# Autodesk Inventor assembly: Tiger
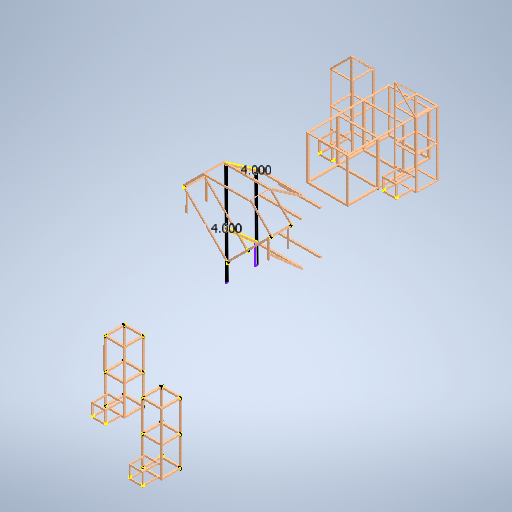
[picture p0: Inventor's stored thumbnail of the model, 512x512]
Saved by Autodesk Inventor 2025 (Build 290162000, 162)
## iProperties
Created: 2024-06-05
Part Number: Tiger
Document SubType Name: Assembly
Designer: Cupri
Mass: 180546 g
Surface Area: 136258 cm^2
Volume: 328266 cm^3
Density: 0.55 g/cm^3
Author: Cupri
## Documents named in this file (38)
- C:\Users\Win\Documents\GitHub\USCTigerBurn24\v2\Tiger.iam
- C:\Users\Win\Documents\GitHub\USCTigerBurn24\Standard Timber\4x4x72.ipt
- C:\Users\Win\Documents\GitHub\USCTigerBurn24\Standard Timber\4x4x40.ipt
- C:\Users\Win\Documents\GitHub\USCTigerBurn24\Standard Timber\2x4x36.ipt
- C:\Users\Win\Documents\GitHub\USCTigerBurn24\Standard Timber\2x4x40.ipt
- C:\Users\Win\Documents\GitHub\USCTigerBurn24\Standard Timber\2x4x24.ipt
- C:\Users\Win\Documents\GitHub\USCTigerBurn24\Standard Timber\2x4x28.ipt
- C:\Users\Win\Documents\GitHub\USCTigerBurn24\Standard Timber\2x4x72 (45 90).ipt
- C:\Users\Win\Documents\GitHub\USCTigerBurn24\Standard Timber\2x4x68 (45 90).ipt
- C:\Users\Win\Documents\GitHub\USCTigerBurn24\Standard Timber\2x4x42.343 (45 90).ipt
- C:\Users\Win\Documents\GitHub\USCTigerBurn24\Standard Timber\2x4x72 (30 90).ipt
- C:\Users\Win\Documents\GitHub\USCTigerBurn24\Standard Timber\2x4x44.ipt
- C:\Users\Win\Documents\GitHub\USCTigerBurn24\Standard Timber\4x4x104.303.ipt
- C:\Users\Win\Documents\GitHub\USCTigerBurn24\Standard Timber\4x4xigiveup.ipt
- C:\Users\Win\Documents\GitHub\USCTigerBurn24\Standard Timber\4x4x96.ipt
- C:\Users\Win\Documents\GitHub\USCTigerBurn24\Standard Timber\2x4x96.ipt
- C:\Users\Win\Documents\GitHub\USCTigerBurn24\Standard Timber\2x4xidk.ipt
- C:\Users\Win\Documents\GitHub\USCTigerBurn24\Standard Timber\2x4x120.ipt
- C:\Users\Win\Documents\GitHub\USCTigerBurn24\Standard Timber\2x4x72.ipt
- C:\Users\Win\Documents\GitHub\USCTigerBurn24\Standard Timber\2x4x88.ipt
- C:\Users\Win\Documents\GitHub\USCTigerBurn24\Standard Timber\4x4x55.ipt
- C:\Users\Win\Documents\GitHub\USCTigerBurn24\Standard Timber\4x4x66.ipt
- C:\Users\Win\Documents\GitHub\USCTigerBurn24\Standard Timber\2x4x48.ipt
- C:\Users\Win\Documents\GitHub\USCTigerBurn24\Standard Timber\leg slant.ipt
- C:\Users\Win\Documents\GitHub\USCTigerBurn24\Standard Timber\Leg slant.2.ipt
- C:\Users\Win\Documents\GitHub\USCTigerBurn24\Standard Timber\2x4x48_MIR.ipt
- C:\Users\Win\Documents\GitHub\USCTigerBurn24\Standard Timber\2x4x72_MIR.ipt
- C:\Users\Win\Documents\GitHub\USCTigerBurn24\Standard Timber\2x4x36_MIR.ipt
- C:\Users\Win\Documents\GitHub\USCTigerBurn24\Standard Timber\2x4x24_MIR.ipt
- C:\Users\Win\Documents\GitHub\USCTigerBurn24\Standard Timber\2x4x28_MIR.ipt
- C:\Users\Win\Documents\GitHub\USCTigerBurn24\Standard Timber\leg slant_MIR.ipt
- C:\Users\Win\Documents\GitHub\USCTigerBurn24\Standard Timber\Leg slant.2_MIR.ipt
- C:\Users\Win\Documents\GitHub\USCTigerBurn24\v2\Tiger\AIP\FEA\epzzwi8io.fins
- C:\Users\Win\Documents\GitHub\USCTigerBurn24\v2\Tiger\AIP\FEA\epzzwi8io.fsat
- C:\Users\Win\Documents\GitHub\USCTigerBurn24\v2\Tiger\AIP\FEA\epzzwi8io.ftes
- C:\Users\Win\Documents\GitHub\USCTigerBurn24\v2\Tiger\AIP\FEA\epzzwi8io.fwiz
- C:\Users\Win\Documents\GitHub\USCTigerBurn24\v2\Tiger\AIP\FEA\epzzwi8jk.fmsh
- C:\Users\Win\Documents\GitHub\USCTigerBurn24\v2\Tiger\AIP\FEA\epzzwi8jl.fres
## Components (186 placed, 31 different names)
1. 4x4x104.303:1 — Flush:221, Flush:222
2. 4x4x104.303:2 — Flush:221, Flush:222
3. 4x4xigiveup:1 — Mate:186
4. 4x4xigiveup:2 — Flush:237, Mate:187, Mate:188
5. 4x4x96:1 — Flush:232
6. 4x4x96:2 — Flush:232
7. 4x4x96:3 — Flush:230
8. 4x4x96:4 — Flush:230
9. 4x4x96:5
10. 2x4x96:1 — Mate:186, Flush:237, Mate:187, Mate:188, Mate:191
11. 2x4xidk:1 — Mate:189, Mate:190, Mate:191, Flush:241
12. 2x4xidk:2 — Mate:192, Flush:240, Flush:241
13. 2x4x72 (45 90):1 — Flush:88
14. 2x4x68 (45 90):1 — Flush:44, Flush:88
15. 2x4x72 (45 90):2 — Flush:48, Mate:48, Flush:51, Mate:49
16. 2x4x72 (45 90):3 — Flush:44, Mate:45, Mate:50, Flush:52, Mate:51
17. 2x4x42.343 (45 90):1 — Flush:48
18. 2x4x42.343 (45 90):2 — Mate:45
19. 2x4x72 (30 90):1 — Mate:48, Flush:51, Mate:49, Flush:70, Flush:238, Mate:192, Flush:240
20. 2x4x72 (30 90):2 — Mate:50, Flush:52, Mate:51, Flush:71, Flush:72
21. 2x4x72 (45 90):4 — Mate:61, Flush:61, Flush:62
22. 2x4x68 (45 90):2 — Mate:61, Flush:61, Flush:62
23. 2x4x72 (45 90):5 — Flush:59, Mate:59, Mate:65, Flush:67, Flush:68
24. 2x4x72 (45 90):6 — Flush:63, Flush:64, Mate:68, Flush:73
25. 2x4x42.343 (45 90):3 — Flush:59, Mate:59
26. 2x4x42.343 (45 90):4 — Flush:63
27. 2x4x72 (30 90):3 — Mate:66, Flush:69, Flush:204, Mate:189
28. 2x4x72 (30 90):4 — Flush:64, Mate:67, Mate:69, Flush:239
29. 2x4x44:1 — Mate:67, Flush:71, Flush:72, Flush:239, Mate:190
30. 2x4x44:2 — Mate:65, Flush:67, Flush:68
31. 2x4x44:3 — Mate:66, Flush:69, Flush:70, Flush:204, Flush:238
32. 2x4x44:4 — Mate:68, Flush:73, Mate:69
33. 4x4x72:65
34. 4x4x72:66
35. 4x4x40:117
36. 4x4x40:118
37. 4x4x40:119
38. 4x4x40:120
39. 4x4x40:121
40. 4x4x40:122
41. 4x4x40:123
42. 4x4x40:124
43. 4x4x72:67
44. 4x4x72:68
45. 4x4x40:125
46. 4x4x40:126
47. 4x4x40:127
48. 2x4x40:7
49. 2x4x36:25
50. 2x4x36:26
51. 2x4x36:27
52. 2x4x36:28
53. 2x4x24:13
54. 2x4x24:14
55. 2x4x28:13
56. 2x4x28:14
57. 4x4x72:69
58. 4x4x72:70
59. 4x4x40:128
60. 4x4x40:129
61. 4x4x40:130
62. 4x4x40:131
63. 4x4x72:71
64. 4x4x72:72
65. 4x4x72:73
66. 4x4x72:74
67. 4x4x40:132
68. 4x4x40:133
69. 4x4x40:134
70. 4x4x40:135
71. 4x4x40:136
72. 4x4x40:137
73. 4x4x40:138
74. 4x4x40:139
75. 4x4x72:75
76. 4x4x72:76
77. 4x4x40:140
78. 4x4x40:141
79. 4x4x40:142
80. 2x4x40:8
81. 2x4x36:29
82. 2x4x36:30
83. 2x4x36:31
84. 2x4x36:32
85. 2x4x24:15
86. 2x4x24:16
87. 2x4x28:15
88. 2x4x28:16
89. 4x4x72:77
90. 4x4x72:78
91. 4x4x40:143
92. 4x4x40:144
93. 4x4x40:145
94. 4x4x40:146
95. 4x4x72:79
96. 4x4x72:80
97. 4x4x96:6 — Mate:293, Flush:350, Flush:351, Mate:301, Flush:367, Flush:368, Flush:390, Flush:528
98. 4x4x96:7 — Mate:293, Flush:350, Flush:351, Mate:294, Flush:352, Flush:353, Flush:393, Mate:316, Flush:405, Mate:318
99. 4x4x96:8 — Mate:294, Flush:352, Flush:353, Flush:365, Flush:366, Mate:300, Flush:531
100. 4x4x96:9 — Flush:361, Flush:362, Mate:298, Flush:384
101. 4x4x96:10 — Flush:396, Mate:314, Flush:397, Flush:399
102. 4x4x96:11 — Flush:363, Mate:299, Flush:364, Flush:398
103. 2x4x120:4 — Flush:361, Flush:362, Mate:298, Mate:301, Flush:367, Flush:368, Mate:303, Flush:371, Flush:372, Flush:383, Mate:309, Flush:385, Mate:310, Flush:386, Flush:387, Mate:311, Flush:389, Mate:312
104. 2x4x120:5 — Flush:363, Mate:299, Flush:364, Flush:365, Flush:366, Mate:300, Mate:302, Flush:369, Flush:370
105. 2x4x72:1 — Mate:302, Flush:369, Flush:370
106. 2x4x72:2 — Mate:303, Flush:371, Flush:372, Mate:306, Flush:377, Flush:378, Flush:391, Mate:313
107. 4x4x96:12 — Mate:306, Flush:377, Flush:378, Flush:392
108. 4x4x96:13 — Flush:403, Flush:404, Flush:406, Mate:317
109. 4x4x96:14
110. 4x4x96:15 — Flush:383, Mate:309, Flush:384, Mate:383
111. 4x4x96:16 — Flush:394, Flush:395, Mate:315, Flush:400, Flush:401
112. 4x4x96:17 — Flush:388
113. 2x4x88:1 — Flush:385, Mate:310, Flush:386
114. 2x4x88:2 — Flush:387, Mate:311, Flush:388
115. 2x4x88:3 — Flush:389, Flush:390, Mate:312
116. 2x4x88:4 — Flush:391, Flush:392, Mate:313
117. 4x4x55:1 — Flush:393, Flush:394, Flush:395
118. 4x4x55:2 — Flush:396, Mate:314, Flush:397, Flush:527
119. 4x4x55:3 — Flush:398, Flush:399, Mate:315, Flush:530
120. 4x4x55:4 — Flush:400, Mate:316, Flush:401, Mate:389
121. 4x4x66:1 — Flush:403, Flush:404, Mate:318
122. 4x4x66:2 — Flush:405, Flush:406, Mate:317
123. 2x4x48:1 — Mate:319, Flush:407, Flush:408, Mate:322, Mate:330, Flush:422, Flush:423
124. 2x4x48:2 — Flush:409, Mate:320, Flush:410, Mate:321, Flush:411, Mate:328, Flush:419, Flush:461, Mate:347, Flush:527
125. 2x4x48:3 — Mate:319, Flush:407, Flush:408, Flush:409, Mate:320, Flush:410, Mate:327, Flush:417, Flush:418
126. 2x4x48:4 — Mate:321, Flush:411, Mate:322, Mate:329, Flush:420, Flush:421
127. 2x4x48:5 — Flush:452
128. 2x4x48:6 — Flush:426, Flush:427
129. 2x4x48:7 — Mate:331, Flush:424, Flush:425, Flush:430, Flush:431, Flush:453, Mate:339
130. 2x4x48:8 — Flush:428, Flush:429
131. 2x4x72:3 — Mate:327, Flush:417, Flush:418, Mate:331, Flush:424, Flush:425, Flush:430, Flush:431
132. 2x4x72:4 — Mate:328, Flush:419, Flush:426, Flush:427, Mate:346, Flush:462
133. 2x4x72:5 — Mate:329, Flush:420, Flush:421, Flush:428, Flush:429, Flush:464, Mate:383
134. 2x4x72:6 — Mate:330, Flush:422, Flush:423
135. 2x4x48:9 — Flush:445, Flush:446
136. 2x4x48:10 — Mate:337, Flush:449, Flush:450
137. 2x4x48:11
138. 2x4x48:12 — Flush:447, Flush:448, Mate:338, Mate:349, Flush:465, Flush:466
139. 2x4x72:7 — Flush:452, Flush:453, Mate:339
140. 2x4x72:8 — Mate:337, Flush:449, Flush:450
141. 2x4x72:9 — Flush:447, Flush:448, Flush:451, Mate:338
142. 2x4x72:10 — Flush:445, Flush:446, Flush:451
143. 2x4x36:33
144. 2x4x36:34 — Flush:463, Flush:464
145. 2x4x36:35 — Mate:348, Mate:390
146. 2x4x36:36 — Flush:461, Mate:347
147. 2x4x24:17 — Flush:528
148. 2x4x24:18 — Mate:390
149. 2x4x28:17
150. 2x4x28:18
151. 2x4x48:13 — Mate:346, Flush:462, Mate:348, Flush:463
152. 2x4x48:14 — Mate:349, Flush:465, Flush:466, Flush:467, Flush:468, Flush:469, Flush:470
153. leg slant:1 — Flush:467, Flush:468
154. Leg slant.2:1 — Flush:469, Flush:470
155. 2x4x48_MIR:1 — Flush:473, Flush:474, Mate:351, Mate:352, Flush:494, Flush:495, Mate:362
156. 2x4x48_MIR:2 — Flush:471, Mate:350, Flush:472, Flush:475, Mate:353, Flush:489, Mate:360, Mate:371, Flush:519
157. 2x4x48_MIR:3 — Flush:471, Mate:350, Flush:472, Flush:473, Flush:474, Mate:351, Flush:485, Flush:486, Mate:359
158. 2x4x48_MIR:4 — Mate:352, Flush:475, Mate:353, Flush:492, Flush:493, Mate:361, Flush:530
159. 2x4x48_MIR:5 — Flush:477, Flush:479, Mate:355, Mate:356, Flush:502
160. 2x4x48_MIR:6 — Mate:354, Flush:476, Flush:478, Flush:480, Mate:357, Flush:487, Flush:488
161. 2x4x48_MIR:7 — Mate:354, Flush:476, Flush:477, Flush:478, Flush:479, Mate:355, Flush:481, Flush:482, Flush:483, Flush:484, Mate:358, Mate:367, Flush:501
162. 2x4x48_MIR:8 — Mate:356, Flush:480, Mate:357, Flush:490, Flush:491
163. 2x4x72_MIR:1 — Flush:481, Flush:482, Flush:483, Flush:484, Mate:358, Flush:485, Flush:486, Mate:359
164. 2x4x72_MIR:2 — Flush:487, Flush:488, Flush:489, Mate:360, Flush:524, Mate:377
165. 2x4x72_MIR:3 — Flush:490, Flush:491, Flush:492, Flush:493, Mate:361, Flush:518, Mate:389
166. 2x4x72_MIR:4 — Flush:494, Flush:495, Mate:362
167. 2x4x48_MIR:9 — Flush:497, Flush:499, Mate:364, Mate:365, Flush:516, Flush:517, Mate:391
168. 2x4x48_MIR:10 — Mate:363, Flush:496, Flush:498, Flush:500, Mate:366, Flush:507, Flush:508, Mate:369, Flush:509, Flush:510, Flush:529, Mate:387
169. 2x4x48_MIR:11 — Mate:363, Flush:496, Flush:497, Flush:498, Flush:499, Mate:364, Flush:503, Flush:504, Flush:505, Mate:368, Flush:506
170. 2x4x48_MIR:12 — Mate:365, Flush:500, Mate:366, Mate:370, Flush:511, Flush:512, Flush:513, Flush:514, Flush:525, Flush:526, Mate:378
171. 2x4x72_MIR:5 — Mate:367, Flush:501, Flush:502, Flush:503, Flush:504, Flush:505, Mate:368, Flush:506
172. 2x4x72_MIR:6 — Flush:507, Flush:508, Mate:369, Flush:509, Flush:510
173. 2x4x72_MIR:7 — Mate:370, Flush:511, Flush:512, Flush:513, Flush:514, Flush:515
174. 2x4x72_MIR:8 — Flush:515, Flush:516, Flush:517
175. 2x4x36_MIR:1 — Flush:522, Mate:375, Rigid:233
176. 2x4x36_MIR:2 — Flush:518, Mate:373, Flush:520, Mate:374, Flush:521, Flush:523
177. 2x4x36_MIR:3 — Mate:372, Mate:376, Rigid:235, Mate:388
178. 2x4x36_MIR:4 — Mate:371, Flush:519, Mate:372, Rigid:234, Rigid:236
179. 2x4x24_MIR:1 — Mate:373, Flush:520, Rigid:233, Flush:531
180. 2x4x24_MIR:2 — Rigid:234, Mate:388
181. 2x4x28_MIR:1 — Mate:374, Flush:521, Rigid:235
182. 2x4x28_MIR:2 — Flush:522, Mate:375, Rigid:236
183. 2x4x48_MIR:13 — Flush:523, Mate:376, Flush:524, Mate:377
184. 2x4x48_MIR:14 — Flush:525, Flush:526, Mate:378, Mate:379, Mate:380, Mate:381, Mate:382, Mate:386
185. leg slant_MIR:1 — Mate:379, Mate:380, Mate:391
186. Leg slant.2_MIR:1 — Mate:381, Mate:382, Mate:386, Flush:529, Mate:387
## Relationships (433: Flush 242, Mate 145, WeldJoint 46)
- Flush:44: 2x4x68 (45 90):1 ↔ 2x4x72 (45 90):3
- Flush:48: 2x4x72 (45 90):2 ↔ 2x4x42.343 (45 90):1
- Mate:45: 2x4x72 (45 90):3 ↔ 2x4x42.343 (45 90):2
- Mate:48: 2x4x72 (45 90):2 ↔ 2x4x72 (30 90):1
- Flush:51: 2x4x72 (45 90):2 ↔ 2x4x72 (30 90):1
- Mate:49: 2x4x72 (45 90):2 ↔ 2x4x72 (30 90):1
- Mate:50: 2x4x72 (45 90):3 ↔ 2x4x72 (30 90):2
- Flush:52: 2x4x72 (45 90):3 ↔ 2x4x72 (30 90):2
- Mate:51: 2x4x72 (45 90):3 ↔ 2x4x72 (30 90):2
- [Flush]: 2x4x68 (45 90):2 ↔ 2x4x72 (45 90):6
- [Flush]: 2x4x72 (45 90):5 ↔ 2x4x42.343 (45 90):3
- [Mate]: 2x4x72 (45 90):6 ↔ 2x4x42.343 (45 90):4
- [Mate]: 2x4x72 (45 90):5 ↔ 2x4x72 (30 90):3
- [Flush]: 2x4x72 (45 90):5 ↔ 2x4x72 (30 90):3
- [Mate]: 2x4x72 (45 90):5 ↔ 2x4x72 (30 90):3
- [Mate]: 2x4x72 (45 90):6 ↔ 2x4x72 (30 90):4
- [Flush]: 2x4x72 (45 90):6 ↔ 2x4x72 (30 90):4
- [Mate]: 2x4x72 (45 90):6 ↔ 2x4x72 (30 90):4
- Flush:59: 2x4x72 (45 90):5 ↔ 2x4x42.343 (45 90):3
- Mate:59: 2x4x72 (45 90):5 ↔ 2x4x42.343 (45 90):3
- Mate:61: 2x4x72 (45 90):4 ↔ 2x4x68 (45 90):2
- Flush:61: 2x4x72 (45 90):4 ↔ 2x4x68 (45 90):2
- Flush:62: 2x4x72 (45 90):4 ↔ 2x4x68 (45 90):2
- Flush:63: 2x4x72 (45 90):6 ↔ 2x4x42.343 (45 90):4
- Flush:64: 2x4x72 (45 90):6 ↔ 2x4x72 (30 90):4
- Mate:65: 2x4x72 (45 90):5 ↔ 2x4x44:2
- Flush:67: 2x4x72 (45 90):5 ↔ 2x4x44:2
- Flush:68: 2x4x72 (45 90):5 ↔ 2x4x44:2
- Mate:66: 2x4x72 (30 90):3 ↔ 2x4x44:3
- Flush:69: 2x4x72 (30 90):3 ↔ 2x4x44:3
- Flush:70: 2x4x72 (30 90):1 ↔ 2x4x44:3
- Mate:67: 2x4x72 (30 90):4 ↔ 2x4x44:1
- Flush:71: 2x4x72 (30 90):2 ↔ 2x4x44:1
- Flush:72: 2x4x72 (30 90):2 ↔ 2x4x44:1
- Mate:68: 2x4x72 (45 90):6 ↔ 2x4x44:4
- Flush:73: 2x4x72 (45 90):6 ↔ 2x4x44:4
- Mate:69: 2x4x72 (30 90):4 ↔ 2x4x44:4
- Flush:88: 2x4x72 (45 90):1 ↔ 2x4x68 (45 90):1
- Flush:204: 2x4x72 (30 90):3 ↔ 2x4x44:3
- Flush:221: 4x4x104.303:1 ↔ 4x4x104.303:2
- Flush:222: 4x4x104.303:1 ↔ 4x4x104.303:2
- Flush:230: 4x4x96:3 ↔ 4x4x96:4
- Flush:232: 4x4x96:1 ↔ 4x4x96:2
- Mate:186: 4x4xigiveup:1 ↔ 2x4x96:1
- Flush:237: 4x4xigiveup:2 ↔ 2x4x96:1
- Mate:187: 4x4xigiveup:2 ↔ 2x4x96:1
- Mate:188: 4x4xigiveup:2 ↔ 2x4x96:1
- Flush:238: 2x4x72 (30 90):1 ↔ 2x4x44:3
- Flush:239: 2x4x72 (30 90):4 ↔ 2x4x44:1
- Mate:189: 2x4xidk:1 ↔ 2x4x72 (30 90):3
- Mate:190: 2x4xidk:1 ↔ 2x4x44:1
- Mate:191: 2x4x96:1 ↔ 2x4xidk:1
- Mate:192: 2x4xidk:2 ↔ 2x4x72 (30 90):1
- Flush:240: 2x4xidk:2 ↔ 2x4x72 (30 90):1
- Flush:241: 2x4xidk:1 ↔ 2x4xidk:2
- [WeldJoint]: 4x4x72:65 ↔ 4x4x40:117
- [WeldJoint]: 4x4x72:66 ↔ 4x4x40:117
- [WeldJoint]: 4x4x72:65 ↔ 4x4x40:118
- [WeldJoint]: 4x4x72:66 ↔ 4x4x40:120
- [WeldJoint]: 4x4x40:118 ↔ 4x4x72:67
- [WeldJoint]: 4x4x40:119 ↔ 4x4x72:67
- [WeldJoint]: 4x4x40:120 ↔ 4x4x72:68
- [WeldJoint]: 4x4x72:66 ↔ 4x4x40:121
- [WeldJoint]: 4x4x40:122 ↔ 4x4x72:67
- [WeldJoint]: 4x4x72:65 ↔ 4x4x40:124
- [WeldJoint]: 4x4x72:65 ↔ 4x4x40:123
- [Mate]: 4x4x72:67 ↔ 2x4x40:7
- [Flush]: 4x4x72:67 ↔ 2x4x40:7
- [Mate] (609.6 mm): 4x4x40:119 ↔ 2x4x40:7
- [Mate] (101.6 mm): 4x4x40:119 ↔ 2x4x36:25
- [Flush]: 4x4x40:119 ↔ 2x4x36:25
- [Mate] (101.6 mm): 4x4x72:68 ↔ 2x4x36:28
- [Flush]: 4x4x40:119 ↔ 2x4x36:28
- [Mate] (101.6 mm): 2x4x40:7 ↔ 2x4x36:26
- [Flush]: 2x4x40:7 ↔ 2x4x36:26
- [Mate]: 2x4x40:7 ↔ 2x4x36:27
- [Flush]: 2x4x40:7 ↔ 2x4x36:27
- [Mate]: 2x4x36:27 ↔ 2x4x36:28
- [WeldJoint]: 2x4x36:25 ↔ 2x4x24:13
- [WeldJoint]: 2x4x36:28 ↔ 2x4x24:14
- [WeldJoint]: 2x4x36:27 ↔ 2x4x28:13
- [WeldJoint]: 2x4x36:28 ↔ 2x4x28:14
- [WeldJoint]: 4x4x72:70 ↔ 4x4x40:128
- [WeldJoint]: 4x4x40:129 ↔ 4x4x72:71
- [WeldJoint]: 4x4x72:69 ↔ 4x4x40:131
- [WeldJoint]: 4x4x72:69 ↔ 4x4x40:130
- [Flush]: 2x4x40:7 ↔ 2x4x36:26
- [Flush]: 2x4x40:7 ↔ 2x4x36:27
- [Flush]: 4x4x40:119 ↔ 2x4x36:25
- [Flush]: 4x4x40:119 ↔ 2x4x36:28
- [Flush] (203.2 mm): 4x4x72:68 ↔ 2x4x36:27
- [Flush] (203.2 mm): 4x4x72:68 ↔ 2x4x36:28
- [Flush]: 2x4x36:25 ↔ 2x4x28:14
- [Mate]: 2x4x36:26 ↔ 2x4x28:13
- [Flush]: 4x4x40:129 ↔ 4x4x72:71
- [Flush]: 4x4x40:129 ↔ 4x4x72:72
- [Mate]: 4x4x40:129 ↔ 4x4x72:72
- [Mate]: 4x4x40:128 ↔ 4x4x72:72
- [Flush]: 4x4x40:128 ↔ 4x4x72:72
- [Flush]: 4x4x72:70 ↔ 4x4x40:128
- [Mate]: 4x4x72:70 ↔ 4x4x40:128
- [Flush]: 4x4x72:69 ↔ 4x4x40:131
- [Flush]: 4x4x72:69 ↔ 4x4x40:130
- [Mate]: 4x4x72:67 ↔ 2x4x40:7
- [Mate]: 2x4x36:26 ↔ 2x4x24:13
- [Flush]: 4x4x72:68 ↔ 4x4x72:72
- [Flush]: 4x4x72:68 ↔ 4x4x72:72
- [WeldJoint]: 4x4x72:73 ↔ 4x4x40:132
- [WeldJoint]: 4x4x72:74 ↔ 4x4x40:132
- [WeldJoint]: 4x4x72:73 ↔ 4x4x40:133
- [WeldJoint]: 4x4x72:74 ↔ 4x4x40:135
- [WeldJoint]: 4x4x40:133 ↔ 4x4x72:75
- [WeldJoint]: 4x4x40:134 ↔ 4x4x72:75
- [WeldJoint]: 4x4x40:135 ↔ 4x4x72:76
- [WeldJoint]: 4x4x72:74 ↔ 4x4x40:136
- [WeldJoint]: 4x4x40:137 ↔ 4x4x72:75
- [WeldJoint]: 4x4x72:73 ↔ 4x4x40:139
- [WeldJoint]: 4x4x72:73 ↔ 4x4x40:138
- [Mate]: 4x4x72:75 ↔ 2x4x40:8
- [Flush]: 4x4x72:75 ↔ 2x4x40:8
- [Mate] (609.6 mm): 4x4x40:134 ↔ 2x4x40:8
- [Mate] (101.6 mm): 4x4x40:134 ↔ 2x4x36:29
- [Flush]: 4x4x40:134 ↔ 2x4x36:29
- [Mate] (101.6 mm): 4x4x72:76 ↔ 2x4x36:32
- [Flush]: 4x4x40:134 ↔ 2x4x36:32
- [Mate]: 2x4x40:8 ↔ 2x4x36:31
- [Flush]: 2x4x40:8 ↔ 2x4x36:31
- [Mate]: 2x4x36:31 ↔ 2x4x36:32
- [WeldJoint]: 2x4x36:29 ↔ 2x4x24:15
- [WeldJoint]: 2x4x36:32 ↔ 2x4x24:16
- [WeldJoint]: 2x4x36:31 ↔ 2x4x28:15
- [WeldJoint]: 2x4x36:32 ↔ 2x4x28:16
- [WeldJoint]: 4x4x72:78 ↔ 4x4x40:143
- [WeldJoint]: 4x4x40:144 ↔ 4x4x72:79
- [WeldJoint]: 4x4x72:77 ↔ 4x4x40:146
- [WeldJoint]: 4x4x72:77 ↔ 4x4x40:145
- [Flush]: 2x4x40:8 ↔ 2x4x36:31
- [Flush]: 4x4x40:134 ↔ 2x4x36:29
- [Flush]: 4x4x40:134 ↔ 2x4x36:32
- [Flush] (203.2 mm): 4x4x72:76 ↔ 2x4x36:31
- [Flush] (203.2 mm): 4x4x72:76 ↔ 2x4x36:32
- [Flush]: 2x4x36:29 ↔ 2x4x28:16
- [Flush]: 2x4x36:30 ↔ 2x4x28:15
- [Mate]: 2x4x36:30 ↔ 2x4x28:15
- [Flush]: 4x4x40:144 ↔ 4x4x72:79
- [Flush]: 4x4x40:144 ↔ 4x4x72:80
- [Mate]: 4x4x40:144 ↔ 4x4x72:79
- [Mate]: 4x4x40:146 ↔ 4x4x72:79
- [Mate]: 4x4x72:74 ↔ 4x4x72:78
- [Mate]: 4x4x72:75 ↔ 2x4x40:8
- [Mate]: 2x4x40:8 ↔ 2x4x24:15
- [Flush]: 2x4x36:31 ↔ 2x4x24:16
- [Flush]: 2x4x36:31 ↔ 2x4x24:16
- [Mate]: 2x4x40:8 ↔ 2x4x36:30
- [Flush]: 2x4x36:30 ↔ 2x4x28:15
- [Flush]: 2x4x36:30 ↔ 2x4x28:15
- [Mate]: 4x4x72:78 ↔ 4x4x40:145
- Mate:293: 4x4x96:6 ↔ 4x4x96:7
- Flush:350: 4x4x96:6 ↔ 4x4x96:7
- Flush:351: 4x4x96:6 ↔ 4x4x96:7
- Mate:294: 4x4x96:7 ↔ 4x4x96:8
- Flush:352: 4x4x96:7 ↔ 4x4x96:8
- Flush:353: 4x4x96:7 ↔ 4x4x96:8
- [Mate]: 4x4x96:9 ↔ 4x4x96:10
- [Flush]: 4x4x96:9 ↔ 4x4x96:10
- [Flush]: 4x4x96:9 ↔ 4x4x96:10
- [Mate]: 4x4x96:10 ↔ 4x4x96:11
- [Flush]: 4x4x96:10 ↔ 4x4x96:11
- [Flush]: 4x4x96:10 ↔ 4x4x96:11
- Flush:361: 4x4x96:9 ↔ 2x4x120:4
- Flush:362: 4x4x96:9 ↔ 2x4x120:4
- Mate:298: 4x4x96:9 ↔ 2x4x120:4
- Flush:363: 4x4x96:11 ↔ 2x4x120:5
- Mate:299: 4x4x96:11 ↔ 2x4x120:5
- Flush:364: 4x4x96:11 ↔ 2x4x120:5
- Flush:365 (50.8 mm): 4x4x96:8 ↔ 2x4x120:5
- Flush:366: 4x4x96:8 ↔ 2x4x120:5
- Mate:300: 4x4x96:8 ↔ 2x4x120:5
- Mate:301: 4x4x96:6 ↔ 2x4x120:4
- Flush:367: 4x4x96:6 ↔ 2x4x120:4
- Flush:368 (50.8 mm): 4x4x96:6 ↔ 2x4x120:4
- Mate:302: 2x4x120:5 ↔ 2x4x72:1
- Flush:369: 2x4x120:5 ↔ 2x4x72:1
- Flush:370: 2x4x120:5 ↔ 2x4x72:1
- Mate:303: 2x4x120:4 ↔ 2x4x72:2
- Flush:371: 2x4x120:4 ↔ 2x4x72:2
- Flush:372: 2x4x120:4 ↔ 2x4x72:2
- [Mate]: 4x4x96:12 ↔ 4x4x96:13
- [Flush]: 4x4x96:12 ↔ 4x4x96:13
- [Flush]: 4x4x96:12 ↔ 4x4x96:13
- [Mate]: 4x4x96:13 ↔ 4x4x96:14
- [Flush]: 4x4x96:13 ↔ 4x4x96:14
- [Flush]: 4x4x96:13 ↔ 4x4x96:14
- Mate:306: 2x4x72:2 ↔ 4x4x96:12
- Flush:377: 2x4x72:2 ↔ 4x4x96:12
- Flush:378: 2x4x72:2 ↔ 4x4x96:12
- [Mate]: 4x4x96:15 ↔ 4x4x96:16
- [Flush]: 4x4x96:15 ↔ 4x4x96:16
- [Flush]: 4x4x96:15 ↔ 4x4x96:16
- [Mate]: 4x4x96:16 ↔ 4x4x96:17
- [Flush]: 4x4x96:16 ↔ 4x4x96:17
- [Flush]: 4x4x96:16 ↔ 4x4x96:17
- Flush:383: 2x4x120:4 ↔ 4x4x96:15
- Mate:309: 2x4x120:4 ↔ 4x4x96:15
- Flush:384 (1498.6 mm): 4x4x96:9 ↔ 4x4x96:15
- Flush:385: 2x4x120:4 ↔ 2x4x88:1
- Mate:310: 2x4x120:4 ↔ 2x4x88:1
- Flush:386: 2x4x120:4 ↔ 2x4x88:1
- Flush:387: 2x4x120:4 ↔ 2x4x88:2
- Mate:311: 2x4x120:4 ↔ 2x4x88:2
- Flush:388: 4x4x96:17 ↔ 2x4x88:2
- Flush:389: 2x4x120:4 ↔ 2x4x88:3
- Flush:390: 4x4x96:6 ↔ 2x4x88:3
- Mate:312: 2x4x120:4 ↔ 2x4x88:3
- Flush:391: 2x4x72:2 ↔ 2x4x88:4
- Flush:392: 4x4x96:12 ↔ 2x4x88:4
- Mate:313: 2x4x72:2 ↔ 2x4x88:4
- Flush:393: 4x4x96:7 ↔ 4x4x55:1
- Flush:394: 4x4x96:16 ↔ 4x4x55:1
- Flush:395: 4x4x96:16 ↔ 4x4x55:1
- Flush:396: 4x4x96:10 ↔ 4x4x55:2
- Mate:314: 4x4x96:10 ↔ 4x4x55:2
- Flush:397: 4x4x96:10 ↔ 4x4x55:2
- Flush:398: 4x4x96:11 ↔ 4x4x55:3
- Flush:399: 4x4x96:10 ↔ 4x4x55:3
- Mate:315: 4x4x96:16 ↔ 4x4x55:3
- Flush:400: 4x4x96:16 ↔ 4x4x55:4
- Mate:316: 4x4x96:7 ↔ 4x4x55:4
- Flush:401: 4x4x96:16 ↔ 4x4x55:4
- Flush:403: 4x4x96:13 ↔ 4x4x66:1
- Flush:404: 4x4x96:13 ↔ 4x4x66:1
- Flush:405: 4x4x96:7 ↔ 4x4x66:2
- Flush:406: 4x4x96:13 ↔ 4x4x66:2
- Mate:317: 4x4x96:13 ↔ 4x4x66:2
- Mate:318: 4x4x96:7 ↔ 4x4x66:1
- Mate:319: 2x4x48:1 ↔ 2x4x48:3
- Flush:407: 2x4x48:1 ↔ 2x4x48:3
- Flush:408: 2x4x48:1 ↔ 2x4x48:3
- Flush:409: 2x4x48:2 ↔ 2x4x48:3
- Mate:320: 2x4x48:2 ↔ 2x4x48:3
- Flush:410: 2x4x48:2 ↔ 2x4x48:3
- Mate:321: 2x4x48:2 ↔ 2x4x48:4
- Flush:411: 2x4x48:2 ↔ 2x4x48:4
- Mate:322: 2x4x48:1 ↔ 2x4x48:4
- [Mate]: 2x4x48:5 ↔ 2x4x48:7
- [Flush]: 2x4x48:5 ↔ 2x4x48:7
- [Flush]: 2x4x48:5 ↔ 2x4x48:7
- [Flush]: 2x4x48:6 ↔ 2x4x48:7
- [Mate]: 2x4x48:6 ↔ 2x4x48:7
- [Flush]: 2x4x48:6 ↔ 2x4x48:7
- [Mate]: 2x4x48:6 ↔ 2x4x48:8
- [Flush]: 2x4x48:6 ↔ 2x4x48:8
- [Mate]: 2x4x48:5 ↔ 2x4x48:8
- Mate:327: 2x4x48:3 ↔ 2x4x72:3
- Flush:417: 2x4x48:3 ↔ 2x4x72:3
- Flush:418: 2x4x48:3 ↔ 2x4x72:3
- Mate:328: 2x4x48:2 ↔ 2x4x72:4
- Flush:419: 2x4x48:2 ↔ 2x4x72:4
- Mate:329: 2x4x48:4 ↔ 2x4x72:5
- Flush:420: 2x4x48:4 ↔ 2x4x72:5
- Flush:421: 2x4x48:4 ↔ 2x4x72:5
- Mate:330: 2x4x48:1 ↔ 2x4x72:6
- Flush:422: 2x4x48:1 ↔ 2x4x72:6
- Flush:423: 2x4x48:1 ↔ 2x4x72:6
- Mate:331: 2x4x48:7 ↔ 2x4x72:3
- Flush:424: 2x4x48:7 ↔ 2x4x72:3
- Flush:425: 2x4x48:7 ↔ 2x4x72:3
- Flush:426: 2x4x48:6 ↔ 2x4x72:4
- Flush:427: 2x4x48:6 ↔ 2x4x72:4
- Flush:428: 2x4x48:8 ↔ 2x4x72:5
- Flush:429: 2x4x48:8 ↔ 2x4x72:5
- Flush:430: 2x4x48:7 ↔ 2x4x72:3
- Flush:431: 2x4x48:7 ↔ 2x4x72:3
- [Mate]: 2x4x48:9 ↔ 2x4x48:11
- [Flush]: 2x4x48:9 ↔ 2x4x48:11
- [Flush]: 2x4x48:9 ↔ 2x4x48:11
- [Flush]: 2x4x48:10 ↔ 2x4x48:11
- [Mate]: 2x4x48:10 ↔ 2x4x48:11
- [Flush]: 2x4x48:10 ↔ 2x4x48:11
- [Mate]: 2x4x48:10 ↔ 2x4x48:12
- [Flush]: 2x4x48:10 ↔ 2x4x48:12
- [Mate]: 2x4x48:9 ↔ 2x4x48:12
- [Mate]: 2x4x48:11 ↔ 2x4x72:7
- [Flush]: 2x4x48:11 ↔ 2x4x72:7
- [Flush]: 2x4x48:11 ↔ 2x4x72:7
- [Flush]: 2x4x48:10 ↔ 2x4x72:8
- [Flush]: 2x4x48:10 ↔ 2x4x72:8
- [Flush]: 2x4x48:12 ↔ 2x4x72:9
- [Flush]: 2x4x48:12 ↔ 2x4x72:9
- [Flush]: 2x4x48:11 ↔ 2x4x72:7
- [Flush]: 2x4x48:11 ↔ 2x4x72:7
- Mate:337: 2x4x48:10 ↔ 2x4x72:8
- Flush:445: 2x4x48:9 ↔ 2x4x72:10
- Flush:446: 2x4x48:9 ↔ 2x4x72:10
- Flush:447: 2x4x48:12 ↔ 2x4x72:9
- Flush:448: 2x4x48:12 ↔ 2x4x72:9
- Flush:449: 2x4x48:10 ↔ 2x4x72:8
- Flush:450: 2x4x48:10 ↔ 2x4x72:8
- Flush:451: 2x4x72:9 ↔ 2x4x72:10
- Mate:338: 2x4x48:12 ↔ 2x4x72:9
- Flush:452: 2x4x48:5 ↔ 2x4x72:7
- Flush:453: 2x4x48:7 ↔ 2x4x72:7
- Mate:339: 2x4x48:7 ↔ 2x4x72:7
- [Mate]: 2x4x36:35 ↔ 2x4x36:36
- [WeldJoint]: 2x4x36:33 ↔ 2x4x24:17
- [WeldJoint]: 2x4x36:36 ↔ 2x4x24:18
- [WeldJoint]: 2x4x36:35 ↔ 2x4x28:17
- [WeldJoint]: 2x4x36:36 ↔ 2x4x28:18
- [Flush]: 2x4x36:33 ↔ 2x4x28:18
- [Mate]: 2x4x36:34 ↔ 2x4x28:17
- [Mate]: 2x4x36:34 ↔ 2x4x24:17
- [Mate]: 2x4x36:33 ↔ 2x4x28:18
- [Flush]: 2x4x36:34 ↔ 2x4x24:17
- [Flush]: 2x4x36:34 ↔ 2x4x28:17
- Flush:461: 2x4x48:2 ↔ 2x4x36:36
- Mate:346: 2x4x72:4 ↔ 2x4x48:13
- Flush:462: 2x4x72:4 ↔ 2x4x48:13
- Mate:347: 2x4x48:2 ↔ 2x4x36:36
- Mate:348: 2x4x36:35 ↔ 2x4x48:13
- Flush:463: 2x4x36:34 ↔ 2x4x48:13
- Flush:464 (254 mm): 2x4x72:5 ↔ 2x4x36:34
- Mate:349: 2x4x48:12 ↔ 2x4x48:14
- Flush:465: 2x4x48:12 ↔ 2x4x48:14
- Flush:466: 2x4x48:12 ↔ 2x4x48:14
- Flush:467: 2x4x48:14 ↔ leg slant:1
- Flush:468: 2x4x48:14 ↔ leg slant:1
- Flush:469: 2x4x48:14 ↔ Leg slant.2:1
- Flush:470: 2x4x48:14 ↔ Leg slant.2:1
- Flush:471: 2x4x48_MIR:2 ↔ 2x4x48_MIR:3
- Mate:350: 2x4x48_MIR:2 ↔ 2x4x48_MIR:3
- Flush:472: 2x4x48_MIR:2 ↔ 2x4x48_MIR:3
- Flush:473: 2x4x48_MIR:1 ↔ 2x4x48_MIR:3
- Flush:474: 2x4x48_MIR:1 ↔ 2x4x48_MIR:3
- Mate:351: 2x4x48_MIR:1 ↔ 2x4x48_MIR:3
- Mate:352: 2x4x48_MIR:1 ↔ 2x4x48_MIR:4
- Flush:475: 2x4x48_MIR:2 ↔ 2x4x48_MIR:4
- Mate:353: 2x4x48_MIR:2 ↔ 2x4x48_MIR:4
- Mate:354: 2x4x48_MIR:6 ↔ 2x4x48_MIR:7
- Flush:476: 2x4x48_MIR:6 ↔ 2x4x48_MIR:7
- Flush:477: 2x4x48_MIR:5 ↔ 2x4x48_MIR:7
- Flush:478: 2x4x48_MIR:6 ↔ 2x4x48_MIR:7
- Flush:479: 2x4x48_MIR:5 ↔ 2x4x48_MIR:7
- Mate:355: 2x4x48_MIR:5 ↔ 2x4x48_MIR:7
- Mate:356: 2x4x48_MIR:5 ↔ 2x4x48_MIR:8
- Flush:480: 2x4x48_MIR:6 ↔ 2x4x48_MIR:8
- Mate:357: 2x4x48_MIR:6 ↔ 2x4x48_MIR:8
- Flush:481: 2x4x48_MIR:7 ↔ 2x4x72_MIR:1
- Flush:482: 2x4x48_MIR:7 ↔ 2x4x72_MIR:1
- Flush:483: 2x4x48_MIR:7 ↔ 2x4x72_MIR:1
- Flush:484: 2x4x48_MIR:7 ↔ 2x4x72_MIR:1
- Mate:358: 2x4x48_MIR:7 ↔ 2x4x72_MIR:1
- Flush:485: 2x4x48_MIR:3 ↔ 2x4x72_MIR:1
- Flush:486: 2x4x48_MIR:3 ↔ 2x4x72_MIR:1
- Mate:359: 2x4x48_MIR:3 ↔ 2x4x72_MIR:1
- Flush:487: 2x4x48_MIR:6 ↔ 2x4x72_MIR:2
- Flush:488: 2x4x48_MIR:6 ↔ 2x4x72_MIR:2
- Flush:489: 2x4x48_MIR:2 ↔ 2x4x72_MIR:2
- Mate:360: 2x4x48_MIR:2 ↔ 2x4x72_MIR:2
- Flush:490: 2x4x48_MIR:8 ↔ 2x4x72_MIR:3
- Flush:491: 2x4x48_MIR:8 ↔ 2x4x72_MIR:3
- Flush:492: 2x4x48_MIR:4 ↔ 2x4x72_MIR:3
- Flush:493: 2x4x48_MIR:4 ↔ 2x4x72_MIR:3
- Mate:361: 2x4x48_MIR:4 ↔ 2x4x72_MIR:3
- Flush:494: 2x4x48_MIR:1 ↔ 2x4x72_MIR:4
- Flush:495: 2x4x48_MIR:1 ↔ 2x4x72_MIR:4
- Mate:362: 2x4x48_MIR:1 ↔ 2x4x72_MIR:4
- Mate:363: 2x4x48_MIR:10 ↔ 2x4x48_MIR:11
- Flush:496: 2x4x48_MIR:10 ↔ 2x4x48_MIR:11
- Flush:497: 2x4x48_MIR:9 ↔ 2x4x48_MIR:11
- Flush:498: 2x4x48_MIR:10 ↔ 2x4x48_MIR:11
- Flush:499: 2x4x48_MIR:9 ↔ 2x4x48_MIR:11
- Mate:364: 2x4x48_MIR:9 ↔ 2x4x48_MIR:11
- Mate:365: 2x4x48_MIR:9 ↔ 2x4x48_MIR:12
- Flush:500: 2x4x48_MIR:10 ↔ 2x4x48_MIR:12
- Mate:366: 2x4x48_MIR:10 ↔ 2x4x48_MIR:12
- Mate:367: 2x4x48_MIR:7 ↔ 2x4x72_MIR:5
- Flush:501: 2x4x48_MIR:7 ↔ 2x4x72_MIR:5
- Flush:502: 2x4x48_MIR:5 ↔ 2x4x72_MIR:5
- Flush:503: 2x4x48_MIR:11 ↔ 2x4x72_MIR:5
- Flush:504: 2x4x48_MIR:11 ↔ 2x4x72_MIR:5
- Flush:505: 2x4x48_MIR:11 ↔ 2x4x72_MIR:5
- Mate:368: 2x4x48_MIR:11 ↔ 2x4x72_MIR:5
- Flush:506: 2x4x48_MIR:11 ↔ 2x4x72_MIR:5
- Flush:507: 2x4x48_MIR:10 ↔ 2x4x72_MIR:6
- Flush:508: 2x4x48_MIR:10 ↔ 2x4x72_MIR:6
- Mate:369: 2x4x48_MIR:10 ↔ 2x4x72_MIR:6
- Flush:509: 2x4x48_MIR:10 ↔ 2x4x72_MIR:6
- Flush:510: 2x4x48_MIR:10 ↔ 2x4x72_MIR:6
- Mate:370: 2x4x48_MIR:12 ↔ 2x4x72_MIR:7
- Flush:511: 2x4x48_MIR:12 ↔ 2x4x72_MIR:7
- Flush:512: 2x4x48_MIR:12 ↔ 2x4x72_MIR:7
- Flush:513: 2x4x48_MIR:12 ↔ 2x4x72_MIR:7
- Flush:514: 2x4x48_MIR:12 ↔ 2x4x72_MIR:7
- Flush:515: 2x4x72_MIR:7 ↔ 2x4x72_MIR:8
- Flush:516: 2x4x48_MIR:9 ↔ 2x4x72_MIR:8
- Flush:517: 2x4x48_MIR:9 ↔ 2x4x72_MIR:8
- Flush:518 (254 mm): 2x4x72_MIR:3 ↔ 2x4x36_MIR:2
- Mate:371: 2x4x48_MIR:2 ↔ 2x4x36_MIR:4
- Flush:519: 2x4x48_MIR:2 ↔ 2x4x36_MIR:4
- Mate:372: 2x4x36_MIR:3 ↔ 2x4x36_MIR:4
- Mate:373: 2x4x36_MIR:2 ↔ 2x4x24_MIR:1
- Flush:520: 2x4x36_MIR:2 ↔ 2x4x24_MIR:1
- Mate:374: 2x4x36_MIR:2 ↔ 2x4x28_MIR:1
- Flush:521: 2x4x36_MIR:2 ↔ 2x4x28_MIR:1
- Flush:522: 2x4x36_MIR:1 ↔ 2x4x28_MIR:2
- Mate:375: 2x4x36_MIR:1 ↔ 2x4x28_MIR:2
- Flush:523: 2x4x36_MIR:2 ↔ 2x4x48_MIR:13
- Mate:376: 2x4x36_MIR:3 ↔ 2x4x48_MIR:13
- Flush:524: 2x4x72_MIR:2 ↔ 2x4x48_MIR:13
- Mate:377: 2x4x72_MIR:2 ↔ 2x4x48_MIR:13
- Flush:525: 2x4x48_MIR:12 ↔ 2x4x48_MIR:14
- Flush:526: 2x4x48_MIR:12 ↔ 2x4x48_MIR:14
- Mate:378: 2x4x48_MIR:12 ↔ 2x4x48_MIR:14
- Mate:379: 2x4x48_MIR:14 ↔ leg slant_MIR:1
- Mate:380: 2x4x48_MIR:14 ↔ leg slant_MIR:1
- Mate:381: 2x4x48_MIR:14 ↔ Leg slant.2_MIR:1
- Mate:382: 2x4x48_MIR:14 ↔ Leg slant.2_MIR:1
- Rigid:233 [WeldJoint]: 2x4x36_MIR:1 ↔ 2x4x24_MIR:1
- Rigid:234 [WeldJoint]: 2x4x36_MIR:4 ↔ 2x4x24_MIR:2
- Rigid:235 [WeldJoint]: 2x4x36_MIR:3 ↔ 2x4x28_MIR:1
- Rigid:236 [WeldJoint]: 2x4x36_MIR:4 ↔ 2x4x28_MIR:2
- Mate:383: 4x4x96:15 ↔ 2x4x72:5
- Flush:527: 4x4x55:2 ↔ 2x4x48:2
- Flush:528: 4x4x96:6 ↔ 2x4x24:17
- Mate:386: 2x4x48_MIR:14 ↔ Leg slant.2_MIR:1
- Flush:529: 2x4x48_MIR:10 ↔ Leg slant.2_MIR:1
- Mate:387: 2x4x48_MIR:10 ↔ Leg slant.2_MIR:1
- Mate:388: 2x4x36_MIR:3 ↔ 2x4x24_MIR:2
- Mate:389: 4x4x55:4 ↔ 2x4x72_MIR:3
- Flush:530: 4x4x55:3 ↔ 2x4x48_MIR:4
- Mate:390: 2x4x36:35 ↔ 2x4x24:18
- Flush:531: 4x4x96:8 ↔ 2x4x24_MIR:1
- Mate:391: 2x4x48_MIR:9 ↔ leg slant_MIR:1
## Named parameters: sa_0 = 22241.1, d253_d234 = 0 mm, d254_d240 = 0 mm, d255_d242 = 0 mm, d256_d247 = 0 mm, d257_d248 = 0 mm, d258_d249 = 0 mm, d259_d250 = 0 mm, d260_d251 = 0 mm, d261_d252 = 0 mm, sa_1 = 980.999, d827_d499 = 0 mm, d828_d500 = 0 mm, d829_d326 = 0 mm, d830_d327 = 0 mm, d831_d305 = 0 mm, d832_d306 = 0 mm, d833_d311 = 0 mm, d834_d312 = 0 mm, d835_d313 = 0 mm, d836_d314 = 0 mm, d837_d315 = 0 mm, d838_d316 = 0 mm, d839_d317 = 0 mm, d840_d143 = 0 mm, d841_d144 = 0 mm, d842_d145 = 0 mm, d843_d146 = 0 mm, d844_d147 = 203.2 mm, d845_d148 = 203.2 mm, d846_d149 = 0 mm, d847_d150 = 0 mm, d848_d61 = 0 mm, d849_d62 = 0 mm, d850_d63 = 609.6 mm, d851_d68 = 101.6 mm, d852_d69 = 0 mm, d853_d70 = 101.6 mm, d854_d71 = 0 mm, d855_d72 = 101.6 mm, d856_d73 = 0 mm, d857_d74 = 0 mm, d858_d75 = 0 mm, d859_d76 = 0 mm, d860_d77 = 0 mm, d861_d78 = 0 mm, d862_d79 = 0 mm, d863_d80 = 0 mm, d864_d136_d47_d36 = 0 mm, d865_d137_d48_d37 = 0 mm, d866_d138_d49_d38 = 0 mm, d867_d139_d50_d39 = 0 mm, d868_d31 = 0 mm, d869_d32 = 0 mm, d870_d33 = 0 mm, d871_d34 = 0 mm, d872_d35 = 0 mm, d873_d36 = 0 mm, d874_d37 = 0 mm, d875_d38 = 0 mm, d876_d39 = 0 mm, d877_d29 = 0 mm, d878_d30 = 0 mm, d879_d626 = 0 mm, d880_d319 = 0 mm, d881_d320 = 0 mm, d882_d321 = 0 mm, d883_d322 = 0 mm, d884_d323 = 0 mm, d885_d324 = 0 mm, d886_d325 = 0 mm, d887_d299 = 0 mm, d888_d301 = 0 mm, d889_d309 = 0 mm, d890_d310 = 0 mm, d891_d318 = 0 mm, d892_d245 = 0 mm, d893_d246 = 0 mm, d894_d154_d144 = 0 mm, d895_d155_d145 = 0 mm, d896_d156_d146 = 0 mm, d897_d157_d147 = 203.2 mm, d898_d158_d148 = 203.2 mm, d899_d159_d149 = 0 mm, d900_d168_d136_d47_d36 = 0 mm, d901_d169_d137_d48_d37 = 0 mm, d902_d170_d138_d49_d38 = 0 mm, d903_d171_d139_d50_d39 = 0 mm, d904_d173_d61 = 0 mm, d905_d174_d62 = 0 mm, d906_d175_d63 = 609.6 mm, d907_d176_d68 = 101.6 mm, d908_d177_d69 = 0 mm, d909_d178_d70 = 101.6 mm, d910_d179_d71 = 0 mm, d911_d182_d74 = 0 mm, d912_d183_d75 = 0 mm, d913_d184_d76 = 0 mm, d914_d185_d77 = 0 mm, d915_d186_d78 = 0 mm, d916_d187_d79 = 0 mm, d917_d188_d80 = 0 mm, d918_d190_d31 = 0 mm, d919_d191_d32 = 0 mm, d920_d192_d33 = 0 mm, d921_d193_d34 = 0 mm, d922_d194_d35 = 0 mm, d923_d195_d36 = 0 mm, d924_d196_d37 = 0 mm, d925_d197_d38 = 0 mm, d926_d198_d39 = 0 mm, d927_d210_d29 = 0 mm, d928_d211_d30 = 0 mm, d1008_d999 = 0 mm, d1009_d1000 = 0 mm, d1011_d995 = 0 mm, d1012_d996 = 0 mm, d1013_d997 = 0 mm, d1014_d998 = 0 mm, d1042_d995 = 0 mm, d1043_d996 = 0 mm, d1044_d997 = 0 mm, d1045_d998 = 0 mm, d1046_d999 = 0 mm, d1047_d1000 = 0 mm, d1051_d995 = 0 mm, d1052_d996 = 0 mm, d1053_d997 = 0 mm, d1054_d998 = 0 mm, d1055_d999 = 0 mm, d1056_d1000 = 0 mm, d1102_d1093 = 0 mm, d1103_d1094 = 0 mm, d1104_d1098 = 0 mm, d1105_d1099 = 0 mm, d1106_d1100 = 0 mm, d1107_d1101 = 0 mm, d1108_d1095 = 0 mm, d1109_d1096 = 0 mm, d1110_d1097 = 0 mm, d1131_d1130 = 0 mm, d1132_d1122 = 0 mm, d1133_d1123 = 0 mm, d1134_d1124 = 0 mm, d1135_d1125 = 0 mm, d1136_d1126 = 0 mm, d1137_d1127 = 0 mm, d1138_d1128 = 0 mm, d1139_d1129 = 0 mm, d1140_d1102_d1093 = 0 mm, d1141_d1103_d1094 = 0 mm, d1142_d1104_d1098 = 0 mm, d1143_d1105_d1099 = 0 mm, d1144_d1106_d1100 = 0 mm, d1145_d1107_d1101 = 0 mm, d1146_d1108_d1095 = 0 mm, d1147_d1109_d1096 = 0 mm, d1148_d1110_d1097 = 0 mm, d1161_d772_d512 = 0 mm, d1162_d773_d513 = 0 mm, d1163_d774_d514 = 0 mm, d1164_d778_d437_d327 = 0 mm, d1167_d799_d405_d149 = 0 mm, d1168_d800_d406_d150 = 0 mm, d1173_d812_d418_d76 = 0 mm, d1174_d813_d419_d77 = 0 mm, d1175_d814_d420_d78 = 0 mm, d1176_d815_d421_d79 = 0 mm, d1177_d816_d422_d80 = 0 mm
note: some values were not read from the file. Shown as the stored number, unit unknown: "sa_0", "sa_1".
